# Autodesk Inventor assembly: ARM
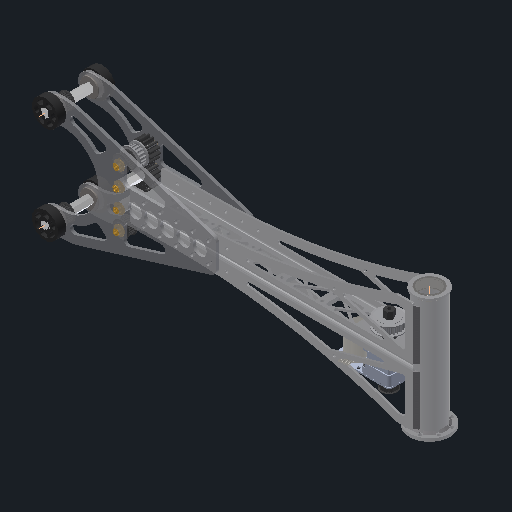
[picture p0: Inventor's stored thumbnail of the model, 512x512]
Saved by Autodesk Inventor 2024.3 (Build 283343000, 343)
## iProperties
Category: _
Manager: _
ILogicPurgeVersion: 0.0.0.0
OnSaveVersion: 3.5.0.0
OnSaveAssembly: COREAutomationManager
Created: 2025-03-17
Part Number: ARM
Checked By: 00
Engr Approved By: _
User Status: Work In Process
Description: ASSY,STANDARD (mm)
Document SubType Name: Assembly
Mfg Approved By: John.Thibert
Designer: John Thibert
Mass: 2242.11 g
Surface Area: 5182.36 cm^2
Volume: 805.847 cm^3
Density: 2.7823 g/cm^3
CN_MASS: 2.24
CN_SERVICEABLE: _
FIRST_DESCRIPTION: _
SECOND_DESCRIPTION: _
THIRD_DESCRIPTION: _
CL_runCount: 0
ModelCat: Uncategorized
Subject: _
Author: John Thibert
Keywords: -
Revision Number: A
## Documents named in this file (15)
- C:\Users\jings\OneDrive\Desktop\FRC 5885\2025-Poseidon-Mechanical\ARM.iam
- C:\Users\jings\OneDrive\Desktop\FRC 5885\2025-Poseidon-Mechanical\WELDMENT,ARM.iam
- C:\Users\jings\OneDrive\Desktop\FRC 5885\2025-Poseidon-Mechanical\180 speed reduced.ipt
- C:\Users\jings\OneDrive\Desktop\FRC 5885\2025-Poseidon-Mechanical\CONTROLS,MOTOR,NEO,550.ipt
- C:\Users\jings\OneDrive\Desktop\FRC 5885\2025-Poseidon-Mechanical\PLATE,END_EFFECTOR,ARM.ipt
- C:\Users\jings\OneDrive\Desktop\FRC 5885\2025-Poseidon-Mechanical\PURCHASED,HEX_BEARING.ipt
- C:\Users\jings\OneDrive\Desktop\FRC 5885\2025-Poseidon-Mechanical\Purchased\5905K518_Needle-Roller Bearing.ipt
- C:\Users\jings\OneDrive\Desktop\FRC 5885\2025-Poseidon-Mechanical\SHAFT,HEX,0.5,WHEELS,ARM.ipt
- C:\Users\jings\OneDrive\Desktop\FRC 5885\2025-Poseidon-Mechanical\1.625 OD Straight Flex Wheel (217-6350)\1.625 OD Straight Flex Wheel (217-6350)\1.625 OD Straight Flex Wheel (217-6350).ipt
- C:\Users\jings\OneDrive\Desktop\FRC 5885\2025-Poseidon-Mechanical\24T x 9mm Wide Double Flange Aluminum Pulley (GT2 3mm, 1_2 Hex Bore) (217-5875)\24T x 9mm Wide Double Flange Aluminum Pulley (GT2 3mm, 1_2 Hex Bore) (217.ipt
- C:\Users\jings\OneDrive\Desktop\FRC 5885\2025-Poseidon-Mechanical\BUSHING,SHAFT,END_EFFECTOR,ARM.ipt
- C:\Users\jings\OneDrive\Desktop\FRC 5885\2025-Poseidon-Mechanical\SHAFT,HEX,0.5,DRIVESHAFT,ARM.ipt
- C:\Users\jings\OneDrive\Desktop\FRC 5885\2025-Poseidon-Mechanical\18T x 9mm Wide Double Flange Aluminum Pulley (HTD 5mm, 1_2” Hex Bore) (217-3225)\18T x 9mm Wide Double Flange Aluminum Pulley (HTD 5mm, 1_2” Hex Bore) (2.ipt
- C:\Users\jings\OneDrive\Desktop\FRC 5885\2025-Poseidon-Mechanical\24T x 9mm Wide Double Flange Aluminum Pulley (HTD 5mm, 1_2” Hex Bore) (217-3227)\24T x 9mm Wide Double Flange Aluminum Pulley (HTD 5mm, 1_2” Hex Bore) (2.ipt
- C:\Users\jings\OneDrive\Desktop\FRC 5885\2025-Poseidon-Mechanical\GEAR,END_EFFECTOR,ARM.ipt
## Components (39 placed, 14 different names)
1. WELDMENT,ARM:1 [sub-assembly] — Mate:2, Mate:11, Mate:12, Mate:13, Flush:2, Flush:3, Mate:14, Mate:15, Mate:16, Mate:17, Mate:18
2. 180 speed reduced:1 — Mate:2, Mate:14, Mate:52, Mate:53
3. CONTROLS,MOTOR,NEO,550:1
4. PURCHASED,HEX_BEARING:3 — Insert:7, Flush:5, Mate:28, Mate:35, Mate:50
5. PURCHASED,HEX_BEARING:1 — Mate:27, Mate:34
6. PURCHASED,HEX_BEARING:2 — Insert:6, Mate:22, Mate:37, Mate:51
7. PURCHASED,HEX_BEARING:4 — Mate:24, Mate:36
8. PLATE,END_EFFECTOR,ARM:2 — Mate:16, Mate:17, Mate:18
9. PLATE,END_EFFECTOR,ARM:3 — Mate:11, Mate:12, Mate:15, Insert:6, Insert:7, Mate:19, Mate:20
10. 5905K518_Needle-Roller Bearing:2
11. 5905K518_Needle-Roller Bearing:1
12. SHAFT,HEX,0.5,WHEELS,ARM:1 — Mate:19, Flush:4, Flush:5, Mate:25, Mate:26, Mate:31, Mate:32, Mate:34, Mate:35, Angle:1, Angle:2
13. SHAFT,HEX,0.5,WHEELS,ARM:2 — Mate:20, Flush:4, Mate:21, Mate:23, Mate:29, Mate:30, Mate:36, Mate:37, Angle:3, Angle:4
14. 1.625 OD Straight Flex Wheel (217-6350):1 — Mate:21, Mate:22, Angle:4
15. 1.625 OD Straight Flex Wheel (217-6350):2 — Mate:23, Mate:24, Angle:3
16. 1.625 OD Straight Flex Wheel (217-6350):3 — Mate:25, Mate:28, Angle:1
17. 1.625 OD Straight Flex Wheel (217-6350):4 — Mate:26, Mate:27, Angle:2
18. 24T x 9mm Wide Double Flange Aluminum Pulley (GT2 3mm, 1_2 Hex Bore) (217:1 — Mate:29, Mate:30, Flush:6, Mate:51, Rotation:5
19. 24T x 9mm Wide Double Flange Aluminum Pulley (GT2 3mm, 1_2 Hex Bore) (217:2 — Mate:31, Mate:32, Flush:7, Mate:50, Rotation:4
20. BUSHING,SHAFT,END_EFFECTOR,ARM:1 — Mate:39
21. BUSHING,SHAFT,END_EFFECTOR,ARM:2 — Mate:44
22. BUSHING,SHAFT,END_EFFECTOR,ARM:3 — Mate:43
23. BUSHING,SHAFT,END_EFFECTOR,ARM:4 — Mate:45
24. BUSHING,SHAFT,END_EFFECTOR,ARM:5 — Mate:38, Mate:61
25. BUSHING,SHAFT,END_EFFECTOR,ARM:6 — Mate:40
26. BUSHING,SHAFT,END_EFFECTOR,ARM:7 — Mate:41
27. BUSHING,SHAFT,END_EFFECTOR,ARM:8 — Mate:42
28. SHAFT,HEX,0.5,DRIVESHAFT,ARM:1 — Mate:38, Mate:39, Mate:46, Mate:47, Mate:54, Mate:55, Mate:57, Mate:58, Rotation:1
29. SHAFT,HEX,0.5,DRIVESHAFT,ARM:2 — Mate:40, Mate:43, Mate:59, Mate:60, Rotation:1, Rotation:2
30. SHAFT,HEX,0.5,DRIVESHAFT,ARM:3 — Mate:41, Mate:44, Mate:62, Mate:63, Rotation:2, Rotation:3
31. SHAFT,HEX,0.5,DRIVESHAFT,ARM:4 — Mate:42, Mate:45, Mate:48, Mate:49, Mate:64, Mate:65, Rotation:3
32. 24T x 9mm Wide Double Flange Aluminum Pulley (GT2 3mm, 1_2 Hex Bore) (217:3 — Mate:46, Mate:47, Flush:7, Mate:56, Rotation:4
33. 24T x 9mm Wide Double Flange Aluminum Pulley (GT2 3mm, 1_2 Hex Bore) (217:4 — Mate:48, Mate:49, Flush:6, Rotation:5
34. 18T x 9mm Wide Double Flange Aluminum Pulley (HTD 5mm, 1_2” Hex Bore) (2:1 — Mate:54, Mate:55, Mate:56
35. 24T x 9mm Wide Double Flange Aluminum Pulley (HTD 5mm, 1_2” Hex Bore) (2:1 — Mate:52, Mate:53
36. Spur Gear1:1 — Mate:57, Mate:58, Mate:61, Flush:8
37. Spur Gear1:2 — Mate:59, Mate:60, Flush:8, Flush:9
38. Spur Gear1:3 — Mate:62, Mate:63, Flush:9, Flush:10
39. Spur Gear1:4 — Mate:64, Mate:65, Flush:10
## Relationships (87: Mate 56, Insert 13, Flush 9, RelateRotation 5, Angle 4)
- [Insert]: 180 speed reduced:1 ↔ CONTROLS,MOTOR,NEO,550:1
- [Mate] (3.175 mm): WELDMENT,ARM:1 ↔ 180 speed reduced:1
- Mate:2: WELDMENT,ARM:1 ↔ 180 speed reduced:1
- [Insert]: PURCHASED,HEX_BEARING:1 ↔ PLATE,END_EFFECTOR,ARM:2
- [Insert]: PURCHASED,HEX_BEARING:4 ↔ PLATE,END_EFFECTOR,ARM:2
- Mate:11: WELDMENT,ARM:1 ↔ PLATE,END_EFFECTOR,ARM:3
- Mate:12: WELDMENT,ARM:1 ↔ PLATE,END_EFFECTOR,ARM:3
- Mate:13: WELDMENT,ARM:1
- Flush:2: WELDMENT,ARM:1
- Flush:3: WELDMENT,ARM:1
- Mate:14: WELDMENT,ARM:1 ↔ 180 speed reduced:1
- Mate:15: WELDMENT,ARM:1 ↔ PLATE,END_EFFECTOR,ARM:3
- Mate:16: WELDMENT,ARM:1 ↔ PLATE,END_EFFECTOR,ARM:2
- Mate:17: WELDMENT,ARM:1 ↔ PLATE,END_EFFECTOR,ARM:2
- Mate:18: WELDMENT,ARM:1 ↔ PLATE,END_EFFECTOR,ARM:2
- Insert:6: PURCHASED,HEX_BEARING:2 ↔ PLATE,END_EFFECTOR,ARM:3
- Insert:7: PURCHASED,HEX_BEARING:3 ↔ PLATE,END_EFFECTOR,ARM:3
- Mate:19: PLATE,END_EFFECTOR,ARM:3 ↔ SHAFT,HEX,0.5,WHEELS,ARM:1
- Mate:20: PLATE,END_EFFECTOR,ARM:3 ↔ SHAFT,HEX,0.5,WHEELS,ARM:2
- Flush:4: SHAFT,HEX,0.5,WHEELS,ARM:1 ↔ SHAFT,HEX,0.5,WHEELS,ARM:2
- Flush:5 (-12.7 mm): PURCHASED,HEX_BEARING:3 ↔ SHAFT,HEX,0.5,WHEELS,ARM:1
- Mate:21: SHAFT,HEX,0.5,WHEELS,ARM:2 ↔ 1.625 OD Straight Flex Wheel (217-6350):1
- Mate:22: PURCHASED,HEX_BEARING:2 ↔ 1.625 OD Straight Flex Wheel (217-6350):1
- Mate:23: SHAFT,HEX,0.5,WHEELS,ARM:2 ↔ 1.625 OD Straight Flex Wheel (217-6350):2
- Mate:24: PURCHASED,HEX_BEARING:4 ↔ 1.625 OD Straight Flex Wheel (217-6350):2
- Mate:25: SHAFT,HEX,0.5,WHEELS,ARM:1 ↔ 1.625 OD Straight Flex Wheel (217-6350):3
- Mate:26: SHAFT,HEX,0.5,WHEELS,ARM:1 ↔ 1.625 OD Straight Flex Wheel (217-6350):4
- Mate:27: PURCHASED,HEX_BEARING:1 ↔ 1.625 OD Straight Flex Wheel (217-6350):4
- Mate:28: PURCHASED,HEX_BEARING:3 ↔ 1.625 OD Straight Flex Wheel (217-6350):3
- Mate:29: SHAFT,HEX,0.5,WHEELS,ARM:2 ↔ 24T x 9mm Wide Double Flange Aluminum Pulley (GT2 3mm, 1_2 Hex Bore) (217:1
- Mate:30: SHAFT,HEX,0.5,WHEELS,ARM:2 ↔ 24T x 9mm Wide Double Flange Aluminum Pulley (GT2 3mm, 1_2 Hex Bore) (217:1
- Mate:31: SHAFT,HEX,0.5,WHEELS,ARM:1 ↔ 24T x 9mm Wide Double Flange Aluminum Pulley (GT2 3mm, 1_2 Hex Bore) (217:2
- Mate:32: SHAFT,HEX,0.5,WHEELS,ARM:1 ↔ 24T x 9mm Wide Double Flange Aluminum Pulley (GT2 3mm, 1_2 Hex Bore) (217:2
- Mate:34: PURCHASED,HEX_BEARING:1 ↔ SHAFT,HEX,0.5,WHEELS,ARM:1
- Mate:35: PURCHASED,HEX_BEARING:3 ↔ SHAFT,HEX,0.5,WHEELS,ARM:1
- Mate:36: PURCHASED,HEX_BEARING:4 ↔ SHAFT,HEX,0.5,WHEELS,ARM:2
- Mate:37: PURCHASED,HEX_BEARING:2 ↔ SHAFT,HEX,0.5,WHEELS,ARM:2
- [Insert]: PLATE,END_EFFECTOR,ARM:3 ↔ BUSHING,SHAFT,END_EFFECTOR,ARM:1
- [Insert]: PLATE,END_EFFECTOR,ARM:3 ↔ BUSHING,SHAFT,END_EFFECTOR,ARM:3
- [Insert]: PLATE,END_EFFECTOR,ARM:3 ↔ BUSHING,SHAFT,END_EFFECTOR,ARM:2
- [Insert]: PLATE,END_EFFECTOR,ARM:3 ↔ BUSHING,SHAFT,END_EFFECTOR,ARM:4
- [Insert]: PLATE,END_EFFECTOR,ARM:2 ↔ BUSHING,SHAFT,END_EFFECTOR,ARM:5
- [Insert]: PLATE,END_EFFECTOR,ARM:2 ↔ BUSHING,SHAFT,END_EFFECTOR,ARM:6
- [Insert]: PLATE,END_EFFECTOR,ARM:2 ↔ BUSHING,SHAFT,END_EFFECTOR,ARM:8
- [Insert]: PLATE,END_EFFECTOR,ARM:2 ↔ BUSHING,SHAFT,END_EFFECTOR,ARM:7
- Mate:38: BUSHING,SHAFT,END_EFFECTOR,ARM:5 ↔ SHAFT,HEX,0.5,DRIVESHAFT,ARM:1
- Mate:39: BUSHING,SHAFT,END_EFFECTOR,ARM:1 ↔ SHAFT,HEX,0.5,DRIVESHAFT,ARM:1
- Mate:40: BUSHING,SHAFT,END_EFFECTOR,ARM:6 ↔ SHAFT,HEX,0.5,DRIVESHAFT,ARM:2
- Mate:41: BUSHING,SHAFT,END_EFFECTOR,ARM:7 ↔ SHAFT,HEX,0.5,DRIVESHAFT,ARM:3
- Mate:42: BUSHING,SHAFT,END_EFFECTOR,ARM:8 ↔ SHAFT,HEX,0.5,DRIVESHAFT,ARM:4
- Mate:43: BUSHING,SHAFT,END_EFFECTOR,ARM:3 ↔ SHAFT,HEX,0.5,DRIVESHAFT,ARM:2
- Mate:44: BUSHING,SHAFT,END_EFFECTOR,ARM:2 ↔ SHAFT,HEX,0.5,DRIVESHAFT,ARM:3
- Mate:45: BUSHING,SHAFT,END_EFFECTOR,ARM:4 ↔ SHAFT,HEX,0.5,DRIVESHAFT,ARM:4
- Mate:46: SHAFT,HEX,0.5,DRIVESHAFT,ARM:1 ↔ 24T x 9mm Wide Double Flange Aluminum Pulley (GT2 3mm, 1_2 Hex Bore) (217:3
- Mate:47: SHAFT,HEX,0.5,DRIVESHAFT,ARM:1 ↔ 24T x 9mm Wide Double Flange Aluminum Pulley (GT2 3mm, 1_2 Hex Bore) (217:3
- Mate:48: SHAFT,HEX,0.5,DRIVESHAFT,ARM:4 ↔ 24T x 9mm Wide Double Flange Aluminum Pulley (GT2 3mm, 1_2 Hex Bore) (217:4
- Mate:49: SHAFT,HEX,0.5,DRIVESHAFT,ARM:4 ↔ 24T x 9mm Wide Double Flange Aluminum Pulley (GT2 3mm, 1_2 Hex Bore) (217:4
- Flush:6: 24T x 9mm Wide Double Flange Aluminum Pulley (GT2 3mm, 1_2 Hex Bore) (217:1 ↔ 24T x 9mm Wide Double Flange Aluminum Pulley (GT2 3mm, 1_2 Hex Bore) (217:4
- Flush:7: 24T x 9mm Wide Double Flange Aluminum Pulley (GT2 3mm, 1_2 Hex Bore) (217:2 ↔ 24T x 9mm Wide Double Flange Aluminum Pulley (GT2 3mm, 1_2 Hex Bore) (217:3
- Mate:50: PURCHASED,HEX_BEARING:3 ↔ 24T x 9mm Wide Double Flange Aluminum Pulley (GT2 3mm, 1_2 Hex Bore) (217:2
- Mate:51: PURCHASED,HEX_BEARING:2 ↔ 24T x 9mm Wide Double Flange Aluminum Pulley (GT2 3mm, 1_2 Hex Bore) (217:1
- Mate:52: 180 speed reduced:1 ↔ 24T x 9mm Wide Double Flange Aluminum Pulley (HTD 5mm, 1_2” Hex Bore) (2:1
- Mate:53: 180 speed reduced:1 ↔ 24T x 9mm Wide Double Flange Aluminum Pulley (HTD 5mm, 1_2” Hex Bore) (2:1
- Mate:54: SHAFT,HEX,0.5,DRIVESHAFT,ARM:1 ↔ 18T x 9mm Wide Double Flange Aluminum Pulley (HTD 5mm, 1_2” Hex Bore) (2:1
- Mate:55: SHAFT,HEX,0.5,DRIVESHAFT,ARM:1 ↔ 18T x 9mm Wide Double Flange Aluminum Pulley (HTD 5mm, 1_2” Hex Bore) (2:1
- Mate:56: 24T x 9mm Wide Double Flange Aluminum Pulley (GT2 3mm, 1_2 Hex Bore) (217:3 ↔ 18T x 9mm Wide Double Flange Aluminum Pulley (HTD 5mm, 1_2” Hex Bore) (2:1
- Mate:57: SHAFT,HEX,0.5,DRIVESHAFT,ARM:1 ↔ Spur Gear1:1
- Mate:58: SHAFT,HEX,0.5,DRIVESHAFT,ARM:1 ↔ Spur Gear1:1
- Mate:59: SHAFT,HEX,0.5,DRIVESHAFT,ARM:2 ↔ Spur Gear1:2
- Mate:60: SHAFT,HEX,0.5,DRIVESHAFT,ARM:2 ↔ Spur Gear1:2
- Mate:61: BUSHING,SHAFT,END_EFFECTOR,ARM:5 ↔ Spur Gear1:1
- Flush:8: Spur Gear1:1 ↔ Spur Gear1:2
- Mate:62: SHAFT,HEX,0.5,DRIVESHAFT,ARM:3 ↔ Spur Gear1:3
- Mate:63: SHAFT,HEX,0.5,DRIVESHAFT,ARM:3 ↔ Spur Gear1:3
- Mate:64: SHAFT,HEX,0.5,DRIVESHAFT,ARM:4 ↔ Spur Gear1:4
- Mate:65: SHAFT,HEX,0.5,DRIVESHAFT,ARM:4 ↔ Spur Gear1:4
- Flush:9: Spur Gear1:2 ↔ Spur Gear1:3
- Flush:10: Spur Gear1:3 ↔ Spur Gear1:4
- Rotation:1 [RelateRotation] (1 ul): SHAFT,HEX,0.5,DRIVESHAFT,ARM:1 ↔ SHAFT,HEX,0.5,DRIVESHAFT,ARM:2
- Rotation:2 [RelateRotation] (1 ul): SHAFT,HEX,0.5,DRIVESHAFT,ARM:2 ↔ SHAFT,HEX,0.5,DRIVESHAFT,ARM:3
- Rotation:3 [RelateRotation] (1 ul): SHAFT,HEX,0.5,DRIVESHAFT,ARM:3 ↔ SHAFT,HEX,0.5,DRIVESHAFT,ARM:4
- Rotation:4 [RelateRotation] (1 ul): 24T x 9mm Wide Double Flange Aluminum Pulley (GT2 3mm, 1_2 Hex Bore) (217:2 ↔ 24T x 9mm Wide Double Flange Aluminum Pulley (GT2 3mm, 1_2 Hex Bore) (217:3
- Angle:1 (0 deg): SHAFT,HEX,0.5,WHEELS,ARM:1 ↔ 1.625 OD Straight Flex Wheel (217-6350):3
- Angle:2 (0 deg): SHAFT,HEX,0.5,WHEELS,ARM:1 ↔ 1.625 OD Straight Flex Wheel (217-6350):4
- Angle:3 (0 deg): SHAFT,HEX,0.5,WHEELS,ARM:2 ↔ 1.625 OD Straight Flex Wheel (217-6350):2
- Angle:4 (0 deg): SHAFT,HEX,0.5,WHEELS,ARM:2 ↔ 1.625 OD Straight Flex Wheel (217-6350):1
- Rotation:5 [RelateRotation] (1 ul): 24T x 9mm Wide Double Flange Aluminum Pulley (GT2 3mm, 1_2 Hex Bore) (217:1 ↔ 24T x 9mm Wide Double Flange Aluminum Pulley (GT2 3mm, 1_2 Hex Bore) (217:4
